# Autodesk Inventor assembly: ASY GBK 1120 long wall shield 2
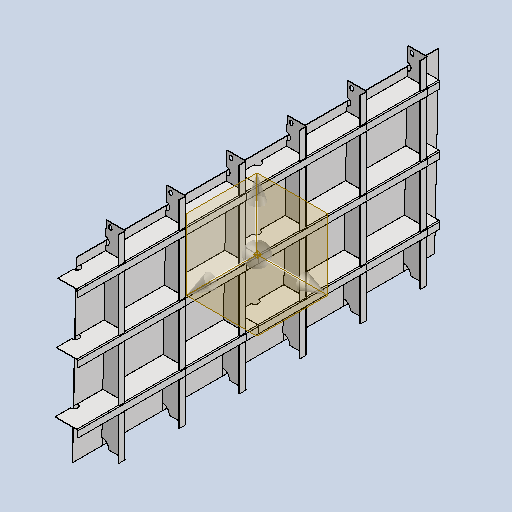
[picture p0: Inventor's stored thumbnail of the model, 512x512]
Saved by Autodesk Inventor 2026.2 (Build 302298010, 298A)
## iProperties
Created: 2026-05-07
Part Number: ASY GBK 1120 long wall shield 2
Document SubType Name: Assembly
Designer: pokla
Mass: 272186 g
Surface Area: 175796 cm^2
Volume: 34673.3 cm^3
Stock Number: 1112
Author: admin
## Documents named in this file (6)
- C:\Users\admin\Documents\Inventor\GBK-Gubkinskiy\ASY GBK 1120 long wall shield 2.iam
- C:\Users\admin\Documents\Inventor\GBK-Gubkinskiy\GBK 0102 stringer 1.ipt
- C:\Users\admin\Documents\Inventor\GBK-Gubkinskiy\GBK 0103 stringer 2.ipt
- C:\Users\admin\Documents\Inventor\GBK-Gubkinskiy\GBK 0104 stringer 3.ipt
- C:\Users\admin\Documents\Inventor\GBK-Gubkinskiy\GBK 0101 main rib.ipt
- C:\Users\admin\Documents\Inventor\GBK-Gubkinskiy\GBK 1125 shield 1.2.ipt
## Components (13 placed, 5 different names)
1. GBK 1125 shield 1.2:1 — Mate:1, Mate:3, Flush:2, Mate:4
2. GBK 0102 stringer 1.ipt:1
3. GBK 0102 stringer 1.ipt:2
4. GBK 0103 stringer 2.ipt:1
5. GBK 0103 stringer 2.ipt:2
6. GBK 0104 stringer 3.ipt:1 — Flush:2
7. GBK 0104 stringer 3.ipt:2
8. GBK 0101 main rib.ipt:1 — Mate:1, Flush:1, Mate:2
9. GBK 0101 main rib.ipt:2
10. GBK 0101 main rib.ipt:3
11. GBK 0101 main rib.ipt:4
12. GBK 0101 main rib.ipt:5
13. GBK 0101 main rib.ipt:6
## Component patterns: (6 elements, first: GBK 0101 main rib.ipt:1)
## Relationships (12: WeldJoint 6, Mate 4, Flush 2)
- [WeldJoint]: GBK 0102 stringer 1.ipt:1 ↔ GBK 0102 stringer 1.ipt:2
- [WeldJoint]: GBK 0103 stringer 2.ipt:1 ↔ GBK 0103 stringer 2.ipt:2
- [WeldJoint]: GBK 0104 stringer 3.ipt:1 ↔ GBK 0104 stringer 3.ipt:2
- [WeldJoint] (4 mm): GBK 0102 stringer 1.ipt:1 ↔ GBK 0101 main rib.ipt:1
- [WeldJoint] (4 mm): GBK 0103 stringer 2.ipt:1 ↔ GBK 0101 main rib.ipt:1
- [WeldJoint] (4 mm): GBK 0104 stringer 3.ipt:1 ↔ GBK 0101 main rib.ipt:1
- Mate:1: GBK 1125 shield 1.2:1 ↔ GBK 0101 main rib.ipt:1
- Flush:1: GBK 0101 main rib.ipt:1
- Mate:2: GBK 0101 main rib.ipt:1
- Mate:3: GBK 1125 shield 1.2:1
- Flush:2 (153 mm): GBK 1125 shield 1.2:1 ↔ GBK 0104 stringer 3.ipt:1
- Mate:4: GBK 1125 shield 1.2:1
## Named parameters: Шаг_шпангоутов = 496.66667 mm
